# Autodesk Inventor assembly: 9P 24T Sprocket, No Insert_MIR
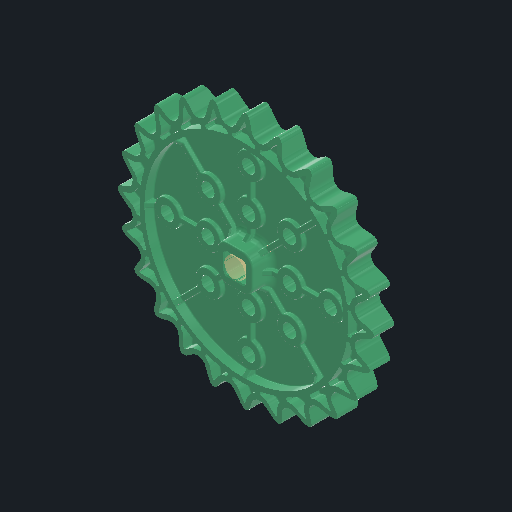
[picture p0: Inventor's stored thumbnail of the model, 512x512]
Saved by Autodesk Inventor 2026.1 (Build 301233000, 233)
## iProperties
Created: 2022-08-02
Part Number: 9P 24T Sprocket, No Insert_MIR
Document SubType Name: Assembly
Designer: roejo
Author: ylu12
## Documents named in this file (2)
- C:\Users\roejo\OneDrive\Documents\3284b-cad-2025\Library\VEX-CAD-Inventor-1.4.2\Motion\Sprockets\9P Sprocket\9P 24T Sprocket, No Insert_MIR.iam
- C:\Users\roejo\OneDrive\Documents\3284b-cad-2025\Library\VEX-CAD-Inventor-1.4.2\Motion\Sprockets\Reference Files\9P 24T Sprocket, No Insert_MIR.ipt
## Components (1 placed, 1 different names)
1. 9P 24T Sprocket, No Insert_MIR:1 — Mate:12, Mate:11, Flush:6
## Relationships (3: Mate 2, Flush 1)
- Mate:12: 9P 24T Sprocket, No Insert_MIR:1
- Mate:11: 9P 24T Sprocket, No Insert_MIR:1
- Flush:6: 9P 24T Sprocket, No Insert_MIR:1
